# Autodesk Inventor assembly: Funnel Assembly
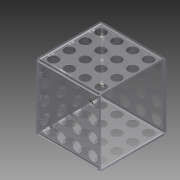
[picture p0: Inventor's stored thumbnail of the model, 180x180]
Saved by Autodesk Inventor 2014 SP1 (Build 180222100, 222)
## iProperties
Created: 2014-01-05
Part Number: Funnel Assembly
Document SubType Name: Assembly
Designer: Michael
Author: Michael
## Documents named in this file (5)
- C:\Users\Arpan\Documents\GitHub\2014buildCAD\Funnel Catcher\Funnel Assembly.iam
- C:\Users\Arpan\Documents\GitHub\2014buildCAD\Funnel Catcher\Funnel Plate Assembly.iam
- C:\Users\Arpan\Documents\GitHub\2014buildCAD\Funnel Catcher\Plastic Funnel PIece.ipt
- C:\Users\Arpan\Documents\GitHub\2014buildCAD\Funnel Catcher\Flange for 3-4 in Piston.ipt
- C:\Users\Arpan\Documents\GitHub\2014buildCAD\Funnel Catcher\9-16 in Pneumatic Cylinder (3 in Stroke).iam
## Components (7 placed, 4 different names)
1. Funnel Plate Assembly:1 [sub-assembly] — Mate:1, Flush:2, Mate:7
2. Funnel Plate Assembly:2 [sub-assembly] — Mate:9, Mate:10, Flush:5
3. Funnel Plate Assembly:3 [sub-assembly] — Mate:3, Mate:6, Mate:8, Flush:3, Mate:10, Flush:4
4. Funnel Plate Assembly:4 [sub-assembly] — Mate:4, Mate:5, Flush:1
5. Plastic Funnel PIece:1 — Mate:1, Mate:3, Mate:4, Mate:5, Mate:6, Flush:1, Flush:2, Mate:7, Mate:8, Flush:3, Mate:9, Mate:11
6. Flange for 3-4 in Piston:1 — Mate:11, Flush:4, Flush:5, Insert:1, Insert:2
7. 9-16 in Pneumatic Cylinder (3 in Stroke):1 [sub-assembly] — Insert:1, Insert:2
## Relationships (17: Mate 10, Flush 5, Insert 2)
- Mate:1: Funnel Plate Assembly:1 ↔ Plastic Funnel PIece:1
- Mate:3: Funnel Plate Assembly:3 ↔ Plastic Funnel PIece:1
- Mate:4: Funnel Plate Assembly:4 ↔ Plastic Funnel PIece:1
- Mate:5: Funnel Plate Assembly:4 ↔ Plastic Funnel PIece:1
- Mate:6: Funnel Plate Assembly:3 ↔ Plastic Funnel PIece:1
- Flush:1: Funnel Plate Assembly:4 ↔ Plastic Funnel PIece:1
- Flush:2: Funnel Plate Assembly:1 ↔ Plastic Funnel PIece:1
- Mate:7: Funnel Plate Assembly:1 ↔ Plastic Funnel PIece:1
- Mate:8: Funnel Plate Assembly:3 ↔ Plastic Funnel PIece:1
- Flush:3: Funnel Plate Assembly:3 ↔ Plastic Funnel PIece:1
- Mate:9: Funnel Plate Assembly:2 ↔ Plastic Funnel PIece:1
- Mate:10: Funnel Plate Assembly:2 ↔ Funnel Plate Assembly:3
- Mate:11: Plastic Funnel PIece:1 ↔ Flange for 3-4 in Piston:1
- Flush:4 (228.6 mm): Funnel Plate Assembly:3 ↔ Flange for 3-4 in Piston:1
- Flush:5 (228.6 mm): Funnel Plate Assembly:2 ↔ Flange for 3-4 in Piston:1
- Insert:1: Flange for 3-4 in Piston:1 ↔ 9-16 in Pneumatic Cylinder (3 in Stroke):1
- Insert:2: Flange for 3-4 in Piston:1 ↔ 9-16 in Pneumatic Cylinder (3 in Stroke):1
